# Autodesk Inventor assembly: Frame
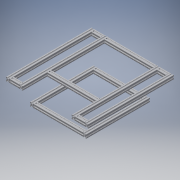
[picture p0: Inventor's stored thumbnail of the model, 180x180]
Saved by Autodesk Inventor 2017 (Build 210142000, 142)
## iProperties
Created: 2018-04-25
Part Number: Frame
Document SubType Name: Assembly
Designer: User
Author: User
## Documents named in this file (5)
- C:\Robotics\CAD\2018-19_CAD\Offseason\Frame.iam
- C:\Robotics\CAD\COTSParts\Bosch Extrusion\Bosch 20x20 17.5 in.ipt
- C:\Robotics\CAD\COTSParts\Bosch Extrusion\Bosch 20x20 1.875in.ipt
- C:\Robotics\CAD\COTSParts\Bosch Extrusion\Bosch 20x20 10in.ipt
- C:\Robotics\CAD\COTSParts\Bosch Extrusion\Bosch 20x20 13 in - Real.ipt
## Components (14 placed, 4 different names)
1. Bosch 20x20 17.5 in:1 — Flush:2, Flush:3, Mate:5, Flush:9, Mate:7, Flush:12, Mate:9, Flush:18, Flush:19, Mate:10, Flush:21, Flush:22, Flush:23, Flush:24, Flush:30
2. Bosch 20x20 17.5 in:2 — Flush:1, Flush:2, Mate:6, Flush:10, Mate:8, Flush:11
3. Bosch 20x20 17.5 in:3 — Flush:3, Flush:4, Mate:2, Flush:8, Mate:4, Flush:17, Mate:11, Flush:20, Mate:12, Flush:25, Flush:26, Flush:29
4. Bosch 20x20 17.5 in:4 — Flush:4, Flush:5, Flush:6, Flush:7, Mate:1, Mate:3
5. Bosch 20x20 1.875in:1 — Flush:1, Mate:3, Mate:4, Flush:17
6. Bosch 20x20 1.875in:2 — Mate:7, Mate:8, Flush:11, Flush:12
7. Bosch 20x20 1.875in:3 — Flush:6, Mate:5, Mate:6, Flush:9, Flush:10
8. Bosch 20x20 1.875in:4 — Flush:5, Flush:7, Mate:1, Mate:2, Flush:8
9. Bosch 20x20 10in:1 — Flush:19, Mate:10, Mate:12, Flush:21
10. Bosch 20x20 10in:2 — Mate:9, Flush:18, Mate:11, Flush:20, Flush:30
11. Bosch 20x20 13 in - Real:1 — Flush:22, Flush:23, Flush:24
12. Bosch 20x20 13 in - Real:2 — Flush:25, Flush:26, Mate:13, Flush:27, Flush:28, Flush:29, Mate:14, Flush:31, Flush:32
13. Bosch 20x20 10in:3 — Mate:13, Flush:27, Flush:28
14. Bosch 20x20 10in:4 — Mate:14, Flush:31, Flush:32
## Relationships (42: Flush 28, Mate 14)
- Flush:1: Bosch 20x20 17.5 in:2 ↔ Bosch 20x20 1.875in:1
- Flush:2: Bosch 20x20 17.5 in:1 ↔ Bosch 20x20 17.5 in:2
- Flush:3: Bosch 20x20 17.5 in:1 ↔ Bosch 20x20 17.5 in:3
- Flush:4: Bosch 20x20 17.5 in:3 ↔ Bosch 20x20 17.5 in:4
- Flush:5: Bosch 20x20 17.5 in:4 ↔ Bosch 20x20 1.875in:4
- Flush:6: Bosch 20x20 17.5 in:4 ↔ Bosch 20x20 1.875in:3
- Flush:7: Bosch 20x20 17.5 in:4 ↔ Bosch 20x20 1.875in:4
- Mate:1: Bosch 20x20 17.5 in:4 ↔ Bosch 20x20 1.875in:4
- Mate:2: Bosch 20x20 17.5 in:3 ↔ Bosch 20x20 1.875in:4
- Flush:8: Bosch 20x20 17.5 in:3 ↔ Bosch 20x20 1.875in:4
- Mate:3: Bosch 20x20 17.5 in:4 ↔ Bosch 20x20 1.875in:1
- Mate:4: Bosch 20x20 17.5 in:3 ↔ Bosch 20x20 1.875in:1
- Mate:5: Bosch 20x20 17.5 in:1 ↔ Bosch 20x20 1.875in:3
- Mate:6: Bosch 20x20 17.5 in:2 ↔ Bosch 20x20 1.875in:3
- Flush:9: Bosch 20x20 17.5 in:1 ↔ Bosch 20x20 1.875in:3
- Flush:10: Bosch 20x20 17.5 in:2 ↔ Bosch 20x20 1.875in:3
- Mate:7: Bosch 20x20 17.5 in:1 ↔ Bosch 20x20 1.875in:2
- Mate:8: Bosch 20x20 17.5 in:2 ↔ Bosch 20x20 1.875in:2
- Flush:11: Bosch 20x20 17.5 in:2 ↔ Bosch 20x20 1.875in:2
- Flush:12: Bosch 20x20 17.5 in:1 ↔ Bosch 20x20 1.875in:2
- Flush:17: Bosch 20x20 17.5 in:3 ↔ Bosch 20x20 1.875in:1
- Mate:9: Bosch 20x20 17.5 in:1 ↔ Bosch 20x20 10in:2
- Flush:18: Bosch 20x20 17.5 in:1 ↔ Bosch 20x20 10in:2
- Flush:19: Bosch 20x20 17.5 in:1 ↔ Bosch 20x20 10in:1
- Mate:10: Bosch 20x20 17.5 in:1 ↔ Bosch 20x20 10in:1
- Mate:11: Bosch 20x20 17.5 in:3 ↔ Bosch 20x20 10in:2
- Flush:20: Bosch 20x20 17.5 in:3 ↔ Bosch 20x20 10in:2
- Mate:12: Bosch 20x20 17.5 in:3 ↔ Bosch 20x20 10in:1
- Flush:21 (127 mm): Bosch 20x20 17.5 in:1 ↔ Bosch 20x20 10in:1
- Flush:22: Bosch 20x20 17.5 in:1 ↔ Bosch 20x20 13 in - Real:1
- Flush:23 (-57.15 mm): Bosch 20x20 17.5 in:1 ↔ Bosch 20x20 13 in - Real:1
- Flush:24 (107.95 mm): Bosch 20x20 17.5 in:1 ↔ Bosch 20x20 13 in - Real:1
- Flush:25: Bosch 20x20 17.5 in:3 ↔ Bosch 20x20 13 in - Real:2
- Flush:26 (-57.15 mm): Bosch 20x20 17.5 in:3 ↔ Bosch 20x20 13 in - Real:2
- Mate:13: Bosch 20x20 13 in - Real:2 ↔ Bosch 20x20 10in:3
- Flush:27: Bosch 20x20 13 in - Real:2 ↔ Bosch 20x20 10in:3
- Flush:28: Bosch 20x20 13 in - Real:2 ↔ Bosch 20x20 10in:3
- Flush:29 (107.95 mm): Bosch 20x20 17.5 in:3 ↔ Bosch 20x20 13 in - Real:2
- Flush:30: Bosch 20x20 17.5 in:1 ↔ Bosch 20x20 10in:2
- Mate:14: Bosch 20x20 13 in - Real:2 ↔ Bosch 20x20 10in:4
- Flush:31: Bosch 20x20 13 in - Real:2 ↔ Bosch 20x20 10in:4
- Flush:32: Bosch 20x20 13 in - Real:2 ↔ Bosch 20x20 10in:4
